# Autodesk Inventor assembly: Fan_top
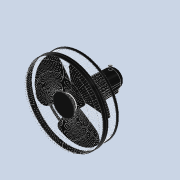
[picture p0: Inventor's stored thumbnail of the model, 180x180]
Saved by Autodesk Inventor 2021 (Build 250183000, 183)
## iProperties
Created: 2020-12-01
Part Number: Fan_top
Document SubType Name: Assembly
Designer: eahil
Author: eahil
## Documents named in this file (6)
- C:\Users\eahil\OneDrive - McMaster University\1P13_IAI\CAD_Labs\Lab 7\Assignment\Fan_Avenue_Version\Fan_top.iam
- C:\Users\eahil\OneDrive - McMaster University\1P13_IAI\CAD_Labs\Lab 7\Assignment\Fan_Avenue_Version\Back Cage.ipt
- C:\Users\eahil\OneDrive - McMaster University\1P13_IAI\CAD_Labs\Lab 7\Assignment\Fan_Avenue_Version\Button.ipt
- C:\Users\eahil\OneDrive - McMaster University\1P13_IAI\CAD_Labs\Lab 7\Assignment\Fan_Avenue_Version\Fan Head.ipt
- C:\Users\eahil\OneDrive - McMaster University\1P13_IAI\CAD_Labs\Lab 7\Assignment\Fan_Avenue_Version\Front Cage.ipt
- C:\Users\eahil\OneDrive - McMaster University\1P13_IAI\CAD_Labs\Lab 7\Assignment\Fan_Avenue_Version\Rotor.ipt
## Components (5 placed, 5 different names)
1. Back Cage:1 — Flush:1, Flush:2, Flush:3, Mate:2, Flush:5, Mate:3, Mate:4, Insert:1
2. Button:1 — Mate:5, Mate:6, Angle:2
3. Fan Head:1 — Flush:4, Mate:2, Flush:5, Mate:5
4. Front Cage:1 — Mate:3, Mate:4, Angle:1
5. Rotor:1 — Insert:1
## Relationships (13: Flush 5, Mate 5, Angle 2, Insert 1)
- Flush:1: Back Cage:1
- Flush:2: Back Cage:1
- Flush:3: Back Cage:1
- Flush:4: Fan Head:1
- Mate:2: Back Cage:1 ↔ Fan Head:1
- Flush:5 (-4 mm): Back Cage:1 ↔ Fan Head:1
- Mate:3: Back Cage:1 ↔ Front Cage:1
- Mate:4: Back Cage:1 ↔ Front Cage:1
- Angle:1 (0 deg): Front Cage:1
- Mate:5: Button:1 ↔ Fan Head:1
- Mate:6 (110 mm): Button:1
- Angle:2 (0 deg): Button:1
- Insert:1 (45 mm): Back Cage:1 ↔ Rotor:1
